# Autodesk Inventor assembly: Desk
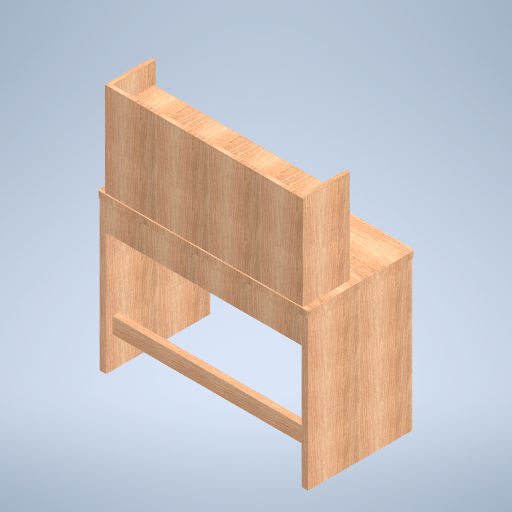
[picture p0: Inventor's stored thumbnail of the model, 512x512]
Saved by Autodesk Inventor 2023 (Build 270158000, 158)
## iProperties
Created: 2022-09-18
Part Number: Desk
Document SubType Name: Assembly
Designer: mliu-23
Author: mliu-23
## Documents named in this file (4)
- D:\MyProfile\Documents\GitHub\VirtualPeddie\CommonObj\CommonObj_Universal\(Desk)CommonObj_Universal_Desk\Desk.iam
- D:\MyProfile\Documents\GitHub\VirtualPeddie\CommonObj\CommonObj_Universal\(Desk)CommonObj_Universal_Desk\Desk.ipt
- D:\MyProfile\Documents\GitHub\VirtualPeddie\CommonObj\CommonObj_Universal\(Desk)CommonObj_Universal_Desk\Drawer.ipt
- D:\MyProfile\Documents\GitHub\VirtualPeddie\CommonObj\CommonObj_Universal\(Desk)CommonObj_Universal_Desk\Shelf.ipt
## Components (3 placed, 3 different names)
1. Desk:1 — Mate:1, Flush:1, Mate:2, Mate:3, Flush:2, Flush:3
2. Drawer:1 — Mate:1, Flush:1, Mate:2
3. Shelf:1 — Mate:3, Flush:2, Flush:3
## Relationships (6: Mate 3, Flush 3)
- Mate:1: Desk:1 ↔ Drawer:1
- Flush:1: Desk:1 ↔ Drawer:1
- Mate:2: Desk:1 ↔ Drawer:1
- Mate:3: Desk:1 ↔ Shelf:1
- Flush:2 (6.35 mm): Desk:1 ↔ Shelf:1
- Flush:3 (25.4 mm): Desk:1 ↔ Shelf:1
